# Autodesk Inventor assembly: PIHTI-for-Boron_2026_non-rotating
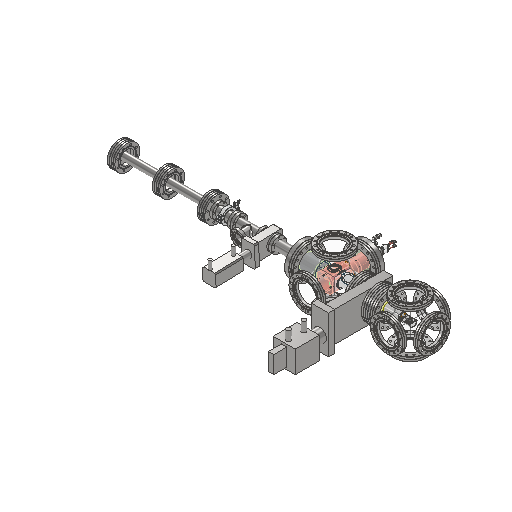
[picture p0: Inventor's stored thumbnail of the model, 512x512]
Saved by Autodesk Inventor 2026.2 (Build 302298000, 298)
## iProperties
Created: 2024-05-09
Part Number: PIHTI-for-Boron_2026_non-rotating
Document SubType Name: Assembly
Designer: kuzmin
Mass: 19614.5 g
Surface Area: 13609.5 cm^2
Volume: 3689.47 cm^3
Density: 5.31636 g/cm^3
Author: kuzmin
## Documents named in this file (25)
- D:\repos\PIHTI\Plasma Vessel_2026\PIHTI-for-Boron_2026_non-rotating.iam
- D:\repos\PIHTI\Plasma Vessel\Plasma-vacuum-cross\Plasma-vacuum-vessel-152IC-cross.iam
- D:\repos\PIHTI\Plasma Vessel\Plasma-Box\Plasma-box-hayashi-aka-upgrade.iam
- D:\repos\PIHTI\ContentCenter\Fastners\M3x8-SHCS.ipt
- D:\repos\PIHTI\Plasma Vessel\Plasma-Box\probe-gate-with-spindel.iam
- D:\repos\PIHTI\Plasma Vessel\Cathode-Anode-Flange\cf70_spacer.ipt
- D:\repos\PIHTI\Plasma Vessel\entrance-mesh-assembly.iam
- D:\repos\PIHTI\Plasma Vessel\probe-port-mesh-welded.iam
- D:\repos\PIHTI\ContentCenter\CF-parts\CF70-nipple\CF70-nipple.iam
- D:\repos\PIHTI\ContentCenter\CF-parts\CF70-gate-valve\Gatevalve_70_pneumatic.iam
- D:\repos\PIHTI\Plasma Vessel_2026\gate_valve\gate_valve_assembly.iam
- D:\repos\PIHTI\Plasma Vessel_2026\Plasma-vacuum-vessel\Plasma-vacuum-vessel-152IC-cross-L205p8.iam
- D:\repos\PIHTI\Plasma Vessel_2026\contents\CF-70-Tee.ipt
- D:\repos\PIHTI\Plasma Vessel_2026\contents\ICF70_to_KF40.ipt
- D:\repos\PIHTI\Plasma Vessel_2026\Cathode-Anode-Flange\Cathode-Anode-70IC-flange-with-feeds.iam
- D:\repos\PIHTI\Plasma Vessel_2026\Plasma-Flange-2024\cathode-box-on-a-flange.iam
- D:\repos\PIHTI\BoronProbe_2026\BoronProbe_2026.iam
- D:\repos\PIHTI\Plasma Vessel_2026\contents\NW40_viton_centering_ring.ipt
- D:\repos\PIHTI\Plasma Vessel_2026\contents\NW40_clamp.ipt
- D:\repos\PIHTI\Plasma Vessel_2026\contents\CF_152-70_bearing.ipt
- D:\repos\PIHTI\Plasma Vessel_2026\contents\M4×12-VentedHexBolt.ipt
- D:\repos\PIHTI\BoronProbe_2026\BoronProbe_2026_non-rotating.iam
- D:\repos\PIHTI\Plasma Vessel_2026\contents\ICF152_bearing_1.ipt
- D:\repos\PIHTI\Plasma Vessel_2026\contents\B_probe_bearing_without_holes.ipt
- D:\repos\PIHTI\BoronProbe_2026\parts\B_probe_bearing.ipt
## Components (35 placed, 23 different names)
1. Plasma-vacuum-vessel-152IC-cross:1 [sub-assembly] — メイト:1, フラッシュ:1, フラッシュ:2, リジッド:18, メイト:22, メイト:23, メイト:24, メイト:59, メイト:60
2. Plasma-box-hayashi-aka-upgrade:1 [sub-assembly] — メイト:3, メイト:4, Hinge Angle, メイト:13, メイト:17
3. probe-gate-with-spindel:1 [sub-assembly] — メイト:3, メイト:4, Hinge Angle
4. cf70_spacer:1 — メイト:61, メイト:62, メイト:63, メイト:64
5. entrance-mesh-assembly:1 [sub-assembly] — メイト:13, メイト:17, メイト:19
6. probe-port-mesh-welded:1 [sub-assembly] — メイト:19
7. CF_152-70_bearing:1 — リジッド:18, リジッド:21, メイト:95, メイト:96, メイト:97
8. CF70-nipple:1 [sub-assembly] — リジッド:21, リジッド:22
9. Gatevalve_70_pneumatic:1 [sub-assembly] — リジッド:22, メイト:47, メイト:48, メイト:49
10. gate_valve_assembly:1 [sub-assembly] — メイト:22, メイト:23, メイト:24, メイト:45, メイト:46, メイト:83, メイト:84, 角度:2
11. Plasma-vacuum-vessel-152IC-cross-L205p8:1 [sub-assembly] — メイト:45, メイト:46, メイト:94
12. CF-70-Tee:1 — メイト:47, メイト:48, メイト:49, メイト:50, メイト:51, メイト:52
13. ICF70_to_KF40:1 — メイト:50, メイト:51, メイト:52, メイト:67, メイト:68, メイト:70, メイト:71
14. Cathode-Anode-70IC-flange-with-feeds:1 [sub-assembly] — メイト:63, メイト:64
15. cathode-box-on-a-flange:1 [sub-assembly] — メイト:59, メイト:60, メイト:61, メイト:62
16. NW40_viton_centering_ring:1 — メイト:67, メイト:68, メイト:81, メイト:82
17. NW40_clamp:1 — メイト:70, メイト:71
18. M4×12-VentedHexBolt:1 — メイト:100, メイト:101
19. M4×12-VentedHexBolt:2 — メイト:98, メイト:99
20. M4×12-VentedHexBolt:3 — メイト:102, メイト:103
21. BoronProbe_2026_non-rotating:1 [sub-assembly] — メイト:81, メイト:82
22. ICF152_bearing_1:1 — メイト:83, メイト:84, 角度:2, メイト:85, メイト:86, メイト:87, メイト:94
23. B_probe_bearing_without_holes:1 — メイト:85, メイト:86, メイト:87, メイト:88, メイト:89, メイト:90, メイト:91, メイト:92, メイト:93
24. M4×12-VentedHexBolt:4 — メイト:88, メイト:89
25. M4×12-VentedHexBolt:5 — メイト:90, メイト:91
26. M4×12-VentedHexBolt:6 — メイト:92, メイト:93
27. B_probe_bearing:1 — メイト:95, メイト:96, メイト:97, メイト:98, メイト:99, メイト:100, メイト:101, メイト:102, メイト:103
28. SS ISO 4762 M3 x 8:5
29. SS ISO 4762 M3 x 8:6
30. SS ISO 4762 M3 x 8:7
31. SS ISO 4762 M3 x 8:8
32. SS ISO 4762 M3 x 8:1
33. SS ISO 4762 M3 x 8:2
34. SS ISO 4762 M3 x 8:3
35. SS ISO 4762 M3 x 8:4
## Relationships (57: Mate 50, WeldJoint 3, Flush 2, Angle 2)
- メイト:1 [Mate]: Plasma-vacuum-vessel-152IC-cross:1
- フラッシュ:1 [Flush]: Plasma-vacuum-vessel-152IC-cross:1
- フラッシュ:2 [Flush]: Plasma-vacuum-vessel-152IC-cross:1
- メイト:3 [Mate]: Plasma-box-hayashi-aka-upgrade:1 ↔ probe-gate-with-spindel:1
- メイト:4 [Mate]: Plasma-box-hayashi-aka-upgrade:1 ↔ probe-gate-with-spindel:1
- Hinge Angle [Angle] (45 deg): Plasma-box-hayashi-aka-upgrade:1 ↔ probe-gate-with-spindel:1
- メイト:13 [Mate]: Plasma-box-hayashi-aka-upgrade:1 ↔ entrance-mesh-assembly:1
- メイト:17 [Mate]: Plasma-box-hayashi-aka-upgrade:1 ↔ entrance-mesh-assembly:1
- メイト:19 [Mate]: entrance-mesh-assembly:1 ↔ probe-port-mesh-welded:1
- リジッド:18 [WeldJoint]: Plasma-vacuum-vessel-152IC-cross:1 ↔ CF_152-70_bearing:1
- リジッド:21 [WeldJoint]: CF_152-70_bearing:1 ↔ CF70-nipple:1
- リジッド:22 [WeldJoint]: CF70-nipple:1 ↔ Gatevalve_70_pneumatic:1
- メイト:22 [Mate]: Plasma-vacuum-vessel-152IC-cross:1 ↔ gate_valve_assembly:1
- メイト:23 [Mate]: Plasma-vacuum-vessel-152IC-cross:1 ↔ gate_valve_assembly:1
- メイト:24 [Mate]: Plasma-vacuum-vessel-152IC-cross:1 ↔ gate_valve_assembly:1
- メイト:45 [Mate]: gate_valve_assembly:1 ↔ Plasma-vacuum-vessel-152IC-cross-L205p8:1
- メイト:46 [Mate]: gate_valve_assembly:1 ↔ Plasma-vacuum-vessel-152IC-cross-L205p8:1
- メイト:47 [Mate]: Gatevalve_70_pneumatic:1 ↔ CF-70-Tee:1
- メイト:48 [Mate]: Gatevalve_70_pneumatic:1 ↔ CF-70-Tee:1
- メイト:49 [Mate]: Gatevalve_70_pneumatic:1 ↔ CF-70-Tee:1
- メイト:50 [Mate]: CF-70-Tee:1 ↔ ICF70_to_KF40:1
- メイト:51 [Mate]: CF-70-Tee:1 ↔ ICF70_to_KF40:1
- メイト:52 [Mate]: CF-70-Tee:1 ↔ ICF70_to_KF40:1
- メイト:59 [Mate]: Plasma-vacuum-vessel-152IC-cross:1 ↔ cathode-box-on-a-flange:1
- メイト:60 [Mate]: Plasma-vacuum-vessel-152IC-cross:1 ↔ cathode-box-on-a-flange:1
- メイト:61 [Mate]: cf70_spacer:1 ↔ cathode-box-on-a-flange:1
- メイト:62 [Mate]: cf70_spacer:1 ↔ cathode-box-on-a-flange:1
- メイト:63 [Mate]: cf70_spacer:1 ↔ Cathode-Anode-70IC-flange-with-feeds:1
- メイト:64 [Mate]: cf70_spacer:1 ↔ Cathode-Anode-70IC-flange-with-feeds:1
- メイト:67 [Mate]: ICF70_to_KF40:1 ↔ NW40_viton_centering_ring:1
- メイト:68 [Mate]: ICF70_to_KF40:1 ↔ NW40_viton_centering_ring:1
- メイト:70 [Mate]: ICF70_to_KF40:1 ↔ NW40_clamp:1
- メイト:71 [Mate]: ICF70_to_KF40:1 ↔ NW40_clamp:1
- メイト:81 [Mate]: NW40_viton_centering_ring:1 ↔ BoronProbe_2026_non-rotating:1
- メイト:82 [Mate]: NW40_viton_centering_ring:1 ↔ BoronProbe_2026_non-rotating:1
- メイト:83 [Mate]: gate_valve_assembly:1 ↔ ICF152_bearing_1:1
- メイト:84 [Mate]: gate_valve_assembly:1 ↔ ICF152_bearing_1:1
- 角度:2 [Angle] (0 deg): gate_valve_assembly:1 ↔ ICF152_bearing_1:1
- メイト:85 [Mate]: ICF152_bearing_1:1 ↔ B_probe_bearing_without_holes:1
- メイト:86 [Mate]: ICF152_bearing_1:1 ↔ B_probe_bearing_without_holes:1
- メイト:87 [Mate]: ICF152_bearing_1:1 ↔ B_probe_bearing_without_holes:1
- メイト:88 [Mate]: B_probe_bearing_without_holes:1 ↔ M4×12-VentedHexBolt:4
- メイト:89 [Mate]: B_probe_bearing_without_holes:1 ↔ M4×12-VentedHexBolt:4
- メイト:90 [Mate]: B_probe_bearing_without_holes:1 ↔ M4×12-VentedHexBolt:5
- メイト:91 [Mate]: B_probe_bearing_without_holes:1 ↔ M4×12-VentedHexBolt:5
- メイト:92 [Mate]: B_probe_bearing_without_holes:1 ↔ M4×12-VentedHexBolt:6
- メイト:93 [Mate]: B_probe_bearing_without_holes:1 ↔ M4×12-VentedHexBolt:6
- メイト:94 [Mate]: Plasma-vacuum-vessel-152IC-cross-L205p8:1 ↔ ICF152_bearing_1:1
- メイト:95 [Mate]: CF_152-70_bearing:1 ↔ B_probe_bearing:1
- メイト:96 [Mate]: CF_152-70_bearing:1 ↔ B_probe_bearing:1
- メイト:97 [Mate]: CF_152-70_bearing:1 ↔ B_probe_bearing:1
- メイト:98 [Mate]: M4×12-VentedHexBolt:2 ↔ B_probe_bearing:1
- メイト:99 [Mate]: M4×12-VentedHexBolt:2 ↔ B_probe_bearing:1
- メイト:100 [Mate]: M4×12-VentedHexBolt:1 ↔ B_probe_bearing:1
- メイト:101 [Mate]: M4×12-VentedHexBolt:1 ↔ B_probe_bearing:1
- メイト:102 [Mate]: M4×12-VentedHexBolt:3 ↔ B_probe_bearing:1
- メイト:103 [Mate]: M4×12-VentedHexBolt:3 ↔ B_probe_bearing:1
## Named parameters: ProbePos = 738 mm
